# Autodesk Inventor assembly: SansRotor
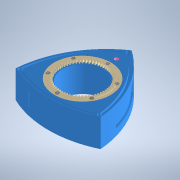
[picture p0: Inventor's stored thumbnail of the model, 180x180]
Saved by Autodesk Inventor 2021 (Build 250183000, 183)
## iProperties
Created: 2021-04-08
Part Number: SansRotor
Document SubType Name: Assembly
Designer: Crist
Author: Crist
## Documents named in this file (4)
- C:\Users\Crist\Desktop\Facultate\CAD\#Proiecte\Wankel_GoleaCristian\SansRotor.iam
- C:\Users\Crist\Desktop\Facultate\CAD\#Proiecte\Wankel_GoleaCristian\Rotor.ipt
- C:\Users\Crist\Desktop\Facultate\CAD\#Proiecte\Wankel_GoleaCristian\Roata.ipt
- C:\Users\Crist\Desktop\Facultate\CAD\#Proiecte\Wankel_GoleaCristian\SubAns-M4.iam
## Components (3 placed, 3 different names)
1. Rotor:1 — Mate:1, Mate:2, Mate:3, Mate:4, Mate:5, Angle:1
2. Roata:1 — Mate:4, Mate:5, Angle:1
3. SubAns-M4:1 [sub-assembly]
## Relationships (7: Mate 5, Angle 1, Insert 1)
- Mate:1: Rotor:1
- Mate:2: Rotor:1
- Mate:3: Rotor:1
- Mate:4: Rotor:1 ↔ Roata:1
- Mate:5: Rotor:1 ↔ Roata:1
- Angle:1 (0 deg): Rotor:1 ↔ Roata:1
- [Insert]: Roata:1 ↔ SubAns-M4:1
